# Autodesk Inventor assembly: HS 48T Gear, Square_MIR
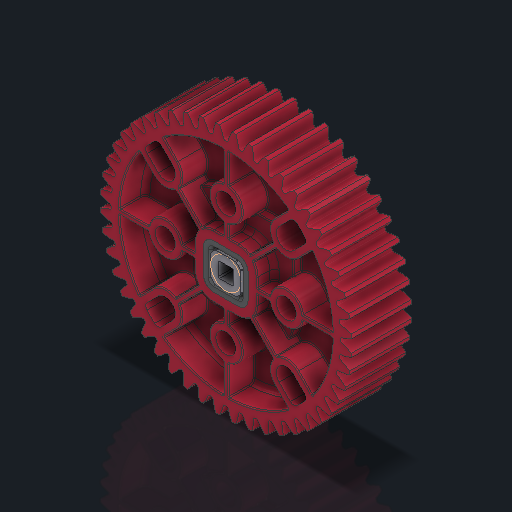
[picture p0: Inventor's stored thumbnail of the model, 512x512]
Saved by Autodesk Inventor 2023.2 (Build 272271030, 271C)
## iProperties
Created: 2022-08-02
Part Number: HS 48T Gear, Square_MIR
Document SubType Name: Assembly
Designer: Michael
Author: ylu12
## Documents named in this file (3)
- C:\Users\black\OneDrive\Pictures\Documents\VEX CAD\VEX-CAD-Inventor-1.4.0\Motion\Gears\HS Gear\HS 48T Gear, Square_MIR.iam
- C:\Users\black\OneDrive\Pictures\Documents\VEX CAD\VEX-CAD-Inventor-1.4.0\Motion\HS Shaft Adapter Square_MIR.ipt
- C:\Users\black\OneDrive\Pictures\Documents\VEX CAD\VEX-CAD-Inventor-1.4.0\Motion\Gears\Reference Files\HS 48T Gear, No Insert_MIR.ipt
## Components (2 placed, 2 different names)
1. HS Shaft Adapter Square_MIR:1 — Flush:2, Mate:4, Mate:3
2. HS 48T Gear, No Insert_MIR:1 — Mate:12, Mate:11, Flush:6
## Relationships (6: Mate 4, Flush 2)
- Flush:2 (-6.35 mm): HS Shaft Adapter Square_MIR:1
- Mate:4: HS Shaft Adapter Square_MIR:1
- Mate:3: HS Shaft Adapter Square_MIR:1
- Mate:12: HS 48T Gear, No Insert_MIR:1
- Mate:11: HS 48T Gear, No Insert_MIR:1
- Flush:6: HS 48T Gear, No Insert_MIR:1
